# Autodesk Inventor assembly: Arm
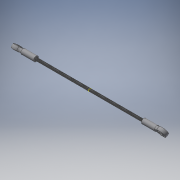
[picture p0: Inventor's stored thumbnail of the model, 180x180]
Saved by Autodesk Inventor 2019.4 (Build 234330000, 330)
## iProperties
Created: 2019-09-26
Part Number: Arm
Document SubType Name: Assembly
Designer: Jorian Bruslind
Author: Jorian Bruslind
## Documents named in this file (3)
- C:\Users\Jorian Bruslind\Documents\GitHub\PersonalProjects\RPI Stellar Photography\Inventor Files\Test Stewart Platform\Arm.iam
- C:\Users\Jorian Bruslind\Documents\GitHub\PersonalProjects\RPI Stellar Photography\Inventor Files\Test Stewart Platform\59935K140_METRIC BALL JOINT ROD END.ipt
- C:\Users\Jorian Bruslind\Documents\GitHub\PersonalProjects\RPI Stellar Photography\Inventor Files\Test Stewart Platform\90024A218_18-8 STAINLESS STEEL THREADED ROD.ipt
## Components (3 placed, 2 different names)
1. 59935K140_METRIC BALL JOINT ROD END:1 — Mate:1, Mate:3
2. 90024A218_18-8 STAINLESS STEEL THREADED ROD:1 — Mate:1, Mate:2, Mate:3, Mate:4
3. 59935K140_METRIC BALL JOINT ROD END:2 — Mate:2, Mate:4
## Relationships (4: Mate 4)
- Mate:1: 59935K140_METRIC BALL JOINT ROD END:1 ↔ 90024A218_18-8 STAINLESS STEEL THREADED ROD:1
- Mate:2: 90024A218_18-8 STAINLESS STEEL THREADED ROD:1 ↔ 59935K140_METRIC BALL JOINT ROD END:2
- Mate:3: 59935K140_METRIC BALL JOINT ROD END:1 ↔ 90024A218_18-8 STAINLESS STEEL THREADED ROD:1
- Mate:4: 90024A218_18-8 STAINLESS STEEL THREADED ROD:1 ↔ 59935K140_METRIC BALL JOINT ROD END:2
